# Autodesk Inventor assembly: calle-pmi
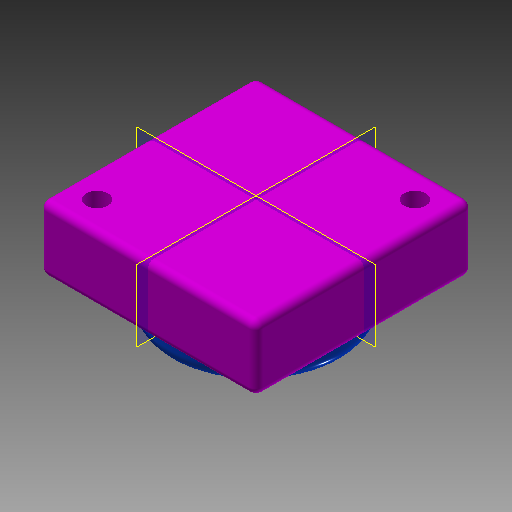
[picture p0: Inventor's stored thumbnail of the model, 512x512]
Saved by Autodesk Inventor 2019 (Build 230136000, 136)
## iProperties
Created: 2020-02-16
Part Number: calle-pmi
Document SubType Name: Assembly
Designer: franc
Author: franc
## Documents named in this file (3)
- C:\Users\franc\Desktop\EsialRobotik\Mecanique\composants\Profile\calle-pmi.iam
- C:\Users\franc\Desktop\EsialRobotik\Mecanique\composants\Profile\patin-teflon-24x5.ipt
- C:\Users\franc\Desktop\EsialRobotik\Mecanique\composants\Profile\calle-patin-pmi.ipt
## Components (2 placed, 2 different names)
1. patin-teflon-24x5:1 — Placage:1, Placage:2, Placage:3
2. calle-patin-pmi:1 — Placage:1, Affleurement:1, Affleurement:2
## Relationships (5: Mate 3, Flush 2)
- Placage:1 [Mate]: patin-teflon-24x5:1 ↔ calle-patin-pmi:1
- Affleurement:1 [Flush] (-15 mm): calle-patin-pmi:1
- Affleurement:2 [Flush] (-15 mm): calle-patin-pmi:1
- Placage:2 [Mate]: patin-teflon-24x5:1
- Placage:3 [Mate]: patin-teflon-24x5:1
